# Autodesk Inventor assembly: TelescopingArm
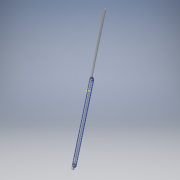
[picture p0: Inventor's stored thumbnail of the model, 180x180]
Saved by Autodesk Inventor 2016 SP1 (Build 200210100, 210)
## iProperties
Created: 2016-01-26
Part Number: TelescopingArm
Document SubType Name: Assembly
Designer: steele
Author: steele
## Documents named in this file (4)
- C:\snobotics\CAD-Development\robSteele\SnoBotics2016\2016-01-31-Lift\TelescopingArm.iam
- C:\snobotics\CAD-Development\robSteele\SnoBotics2016\TelescopeArm\InnerTube.ipt
- C:\snobotics\CAD-Development\robSteele\SnoBotics2016\TelescopeArm\OuterTube.ipt
- C:\snobotics\CAD-Development\robSteele\SnoBotics2016\2016-01-31-Lift\TelescopingArm\Design Accelerator\Chain Drive1.iam
## Components (3 placed, 3 different names)
1. OuterTube:1 — Mate:3, Mate:4, Flush:2
2. InnerTube:1 — Mate:3, Mate:4, Flush:2
3. Chain Drive:1 [sub-assembly]
## Relationships (3: Mate 2, Flush 1)
- Mate:3: OuterTube:1 ↔ InnerTube:1
- Mate:4: OuterTube:1 ↔ InnerTube:1
- Flush:2 (-965.2 mm): OuterTube:1 ↔ InnerTube:1
